# Autodesk Inventor assembly: Robotic_Platform_v0
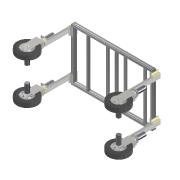
[picture p0: Inventor's stored thumbnail of the model, 180x180]
Saved by Autodesk Inventor 2022 (Build 260153000, 153)
## iProperties
Created: 2024-07-10
Part Number: Robotic_Platform_v0
Document SubType Name: Assembly
Designer: LaptopJR
Author: LaptopJR
## Documents named in this file (12)
- C:\Users\LaptopJR\Documents\Ideation AI\EcoTerrabot\Chassis\CAD files\Robotic_Platform_v0.iam
- C:\Users\LaptopJR\Documents\Ideation AI\EcoTerrabot\Chassis\CAD files\Wheel module\Wheel Module.iam
- C:\Users\LaptopJR\Documents\Ideation AI\EcoTerrabot\Chassis\CAD files\Fixed_Structure\Fixed_Structure.iam
- C:\Users\LaptopJR\Documents\Ideation AI\EcoTerrabot\Chassis\CAD files\LINEAR_BEARING_80_40\657176.iam
- C:\Users\LaptopJR\Documents\Ideation AI\EcoTerrabot\Chassis\CAD files\Fixed_Structure\Leg.iam
- C:\Users\LaptopJR\Documents\Ideation AI\EcoTerrabot\Chassis\CAD files\Fixed_Structure\LegHolder.ipt
- C:\Users\LaptopJR\Documents\Ideation AI\EcoTerrabot\Chassis\CAD files\WheelModuleBracket.ipt
- C:\Users\LaptopJR\Documents\Ideation AI\EcoTerrabot\Chassis\CAD files\Wheel module\Wheel Module_MIR.iam
- C:\Users\LaptopJR\Documents\Ideation AI\EcoTerrabot\Chassis\CAD files\LINEAR_BEARING_80_40\657176_MIR.iam
- C:\Users\LaptopJR\Documents\Ideation AI\EcoTerrabot\Chassis\CAD files\Fixed_Structure\Leg_MIR.iam
- C:\Users\LaptopJR\Documents\Ideation AI\EcoTerrabot\Chassis\CAD files\Fixed_Structure\LegHolder_MIR.ipt
- C:\Users\LaptopJR\Documents\Ideation AI\EcoTerrabot\Chassis\CAD files\WheelModuleBracket_MIR.ipt
## Components (21 placed, 11 different names)
1. Fixed_Structure:1 [sub-assembly] — Mate:1, Mate:2, Mate:3, Mate:16, Mate:17, Flush:8, Mate:20, Mate:21, Mate:32, Mate:33
2. Wheel Module:1 [sub-assembly] — Mate:7, Mate:8, Mate:9
3. Leg:1 [sub-assembly] — Flush:2, Flush:3, Mate:4, Mate:5, Mate:6, Flush:4
4. LegHolder:1 — Flush:1, Flush:2, Flush:3, Mate:4
5. 657176:1 [sub-assembly] — Mate:1, Mate:3, Flush:1
6. WheelModuleBracket:1 — Mate:5, Mate:6, Mate:7, Mate:8, Mate:9, Flush:4
7. Wheel Module_MIR:1 [sub-assembly] — Mate:41, Mate:42, Mate:43
8. Leg_MIR:1 [sub-assembly] — Mate:37, Mate:38, Flush:11, Mate:39, Mate:40, Flush:12
9. LegHolder_MIR:1 — Mate:34, Mate:35, Mate:36, Mate:37, Mate:38, Flush:11
10. 657176_MIR:1 [sub-assembly] — Mate:32, Mate:33, Mate:34, Mate:35, Mate:36
11. WheelModuleBracket_MIR:1 — Mate:39, Mate:40, Flush:12, Mate:41, Mate:42, Mate:43
12. Leg:2 [sub-assembly]
13. LegHolder:2 — Mate:18, Mate:19
14. 657176:2 [sub-assembly] — Mate:16, Mate:17, Mate:18, Mate:19
15. Wheel Module:2 [sub-assembly]
16. WheelModuleBracket:2
17. Leg_MIR:2 [sub-assembly] — Mate:25, Flush:9, Mate:26, Mate:27, Mate:28, Flush:10
18. LegHolder_MIR:2 — Mate:22, Mate:23, Mate:24, Mate:25, Flush:9, Mate:26
19. 657176_MIR:2 [sub-assembly] — Mate:20, Mate:21, Mate:22, Mate:23, Mate:24
20. Wheel Module_MIR:2 [sub-assembly] — Mate:29, Mate:30, Mate:31
21. WheelModuleBracket_MIR:2 — Mate:27, Mate:28, Flush:10, Mate:29, Mate:30, Mate:31
## Relationships (55: Mate 43, Flush 12)
- Mate:1: Fixed_Structure:1 ↔ 657176:1
- Mate:2: Fixed_Structure:1
- Mate:3: Fixed_Structure:1 ↔ 657176:1
- Flush:1: LegHolder:1 ↔ 657176:1
- Flush:2: Leg:1 ↔ LegHolder:1
- Flush:3 (40 mm): Leg:1 ↔ LegHolder:1
- Mate:4: Leg:1 ↔ LegHolder:1
- Mate:5: Leg:1 ↔ WheelModuleBracket:1
- Mate:6: Leg:1 ↔ WheelModuleBracket:1
- Mate:7: Wheel Module:1 ↔ WheelModuleBracket:1
- Mate:8: Wheel Module:1 ↔ WheelModuleBracket:1
- Mate:9: Wheel Module:1 ↔ WheelModuleBracket:1
- Flush:4: Leg:1 ↔ WheelModuleBracket:1
- [Flush]: Leg:2 ↔ LegHolder:2
- [Flush] (40 mm): Leg:2 ↔ LegHolder:2
- [Mate]: Leg:2 ↔ LegHolder:2
- [Mate]: Leg:2 ↔ WheelModuleBracket:2
- [Mate]: Leg:2 ↔ WheelModuleBracket:2
- [Mate]: Wheel Module:2 ↔ WheelModuleBracket:2
- [Mate]: Wheel Module:2 ↔ WheelModuleBracket:2
- [Mate]: Wheel Module:2 ↔ WheelModuleBracket:2
- [Flush]: Leg:2 ↔ WheelModuleBracket:2
- Mate:16: Fixed_Structure:1 ↔ 657176:2
- Mate:17: Fixed_Structure:1 ↔ 657176:2
- Mate:18: LegHolder:2 ↔ 657176:2
- Mate:19: LegHolder:2 ↔ 657176:2
- Flush:8 (-515 mm): Fixed_Structure:1
- Mate:20: Fixed_Structure:1 ↔ 657176_MIR:2
- Mate:21: Fixed_Structure:1 ↔ 657176_MIR:2
- Mate:22: LegHolder_MIR:2 ↔ 657176_MIR:2
- Mate:23: LegHolder_MIR:2 ↔ 657176_MIR:2
- Mate:24: LegHolder_MIR:2 ↔ 657176_MIR:2
- Mate:25: Leg_MIR:2 ↔ LegHolder_MIR:2
- Flush:9: Leg_MIR:2 ↔ LegHolder_MIR:2
- Mate:26: Leg_MIR:2 ↔ LegHolder_MIR:2
- Mate:27: Leg_MIR:2 ↔ WheelModuleBracket_MIR:2
- Mate:28: Leg_MIR:2 ↔ WheelModuleBracket_MIR:2
- Flush:10: Leg_MIR:2 ↔ WheelModuleBracket_MIR:2
- Mate:29: Wheel Module_MIR:2 ↔ WheelModuleBracket_MIR:2
- Mate:30: Wheel Module_MIR:2 ↔ WheelModuleBracket_MIR:2
- Mate:31: Wheel Module_MIR:2 ↔ WheelModuleBracket_MIR:2
- Mate:32: Fixed_Structure:1 ↔ 657176_MIR:1
- Mate:33: Fixed_Structure:1 ↔ 657176_MIR:1
- Mate:34: LegHolder_MIR:1 ↔ 657176_MIR:1
- Mate:35: LegHolder_MIR:1 ↔ 657176_MIR:1
- Mate:36: LegHolder_MIR:1 ↔ 657176_MIR:1
- Mate:37: Leg_MIR:1 ↔ LegHolder_MIR:1
- Mate:38: Leg_MIR:1 ↔ LegHolder_MIR:1
- Flush:11: Leg_MIR:1 ↔ LegHolder_MIR:1
- Mate:39: Leg_MIR:1 ↔ WheelModuleBracket_MIR:1
- Mate:40: Leg_MIR:1 ↔ WheelModuleBracket_MIR:1
- Flush:12: Leg_MIR:1 ↔ WheelModuleBracket_MIR:1
- Mate:41: Wheel Module_MIR:1 ↔ WheelModuleBracket_MIR:1
- Mate:42: Wheel Module_MIR:1 ↔ WheelModuleBracket_MIR:1
- Mate:43: Wheel Module_MIR:1 ↔ WheelModuleBracket_MIR:1
## Named parameters: d16_d7 = 0 mm, d17_d8 = 40 mm, d18_d9 = 0 mm, d19_d10 = 0 mm, d20_d11 = 0 mm, d21_d12 = 0 mm, d22_d13 = 0 mm, d23_d14 = 0 mm, d24_d15 = 0 mm
